# Autodesk Inventor assembly: potteplanteholder
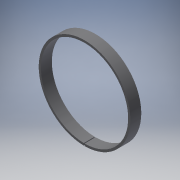
[picture p0: Inventor's stored thumbnail of the model, 180x180]
Saved by Autodesk Inventor 2018 (Build 220112000, 112)
## iProperties
Created: 2019-10-04
Part Number: potteplanteholder
Document SubType Name: Assembly
Designer: gust3763
Author: gust3763
## Documents named in this file (4)
- H:\INVENTOR 2018\WF_navn_2018\DESIGNS\H4\trappe\potteplanteholder\potteplanteholder.iam
- H:\INVENTOR 2018\WF_navn_2018\DESIGNS\H4\trappe\potteplanteholder\hage.ipt
- H:\INVENTOR 2018\WF_navn_2018\DESIGNS\H4\trappe\potteplanteholder\armeringsjern.ipt
- H:\INVENTOR 2018\WF_navn_2018\DESIGNS\H4\trappe\potteplanteholder\valset ring.ipt
## Components (3 placed, 3 different names)
1. hage:1 — Insert:1, Angle:1
2. armeringsjern:1 — Insert:1, Angle:1, Mate:1, Angle:2, Tangent:1
3. valset ring:1 — Mate:1, Angle:2, Tangent:1
## Relationships (5: Angle 2, Insert 1, Mate 1, Tangent 1)
- Insert:1: hage:1 ↔ armeringsjern:1
- Angle:1 (0 deg): hage:1 ↔ armeringsjern:1
- Mate:1: armeringsjern:1 ↔ valset ring:1
- Angle:2 (0 deg): armeringsjern:1 ↔ valset ring:1
- Tangent:1: armeringsjern:1 ↔ valset ring:1
